# Autodesk Inventor assembly: general
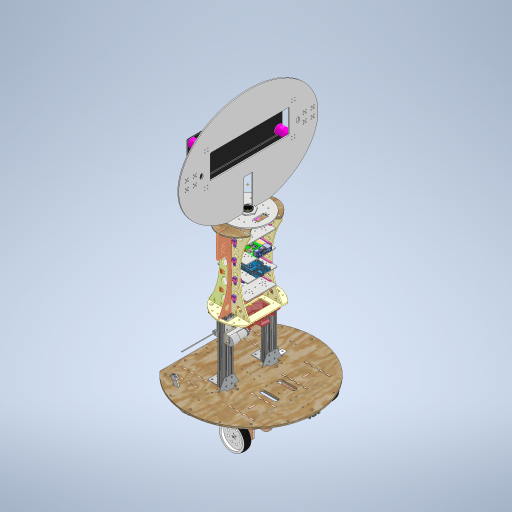
[picture p0: Inventor's stored thumbnail of the model, 512x512]
Saved by Autodesk Inventor 2023.1 (Build 271208000, 208)
## iProperties
Created: 2024-12-19
Part Number: general
Document SubType Name: Assembly
Designer: DELL
Author: DELL
## Documents named in this file (5)
- C:\Users\DELL\reposGitHub\Cheburashka\Cheburashka_construction\general.iam
- C:\Users\DELL\reposGitHub\Cheburashka\Cheburashka_construction\platform\platform.iam
- C:\Users\DELL\reposGitHub\Cheburashka\Cheburashka_construction\korpus\korp.iam
- C:\Users\DELL\reposGitHub\Cheburashka\Cheburashka_construction\platform\8bc17c1464c21f56fb2a3979b7c6b729.ipt
- C:\Users\DELL\reposGitHub\Cheburashka\Cheburashka_construction\face\лицо\Сборка1.iam
## Components (5 placed, 4 different names)
1. platform:1 [sub-assembly] — Заподлицо:1, Совмещение:7, Совмещение:8, Совмещение:13, Совмещение:14
2. korp:1 [sub-assembly] — Заподлицо:1, Совмещение:6, Совмещение:12, Совмещение:15, Совмещение:16, Совмещение:17
3. 8bc17c1464c21f56fb2a3979b7c6b729:2 — Совмещение:6, Совмещение:7, Совмещение:8
4. 8bc17c1464c21f56fb2a3979b7c6b729:4 — Совмещение:12, Совмещение:13, Совмещение:14
5. face [sub-assembly] — Совмещение:15, Совмещение:16, Совмещение:17
## Relationships (10: Mate 9, Flush 1)
- Заподлицо:1 [Flush]: platform:1 ↔ korp:1
- Совмещение:6 [Mate]: korp:1 ↔ 8bc17c1464c21f56fb2a3979b7c6b729:2
- Совмещение:7 [Mate]: platform:1 ↔ 8bc17c1464c21f56fb2a3979b7c6b729:2
- Совмещение:8 [Mate]: platform:1 ↔ 8bc17c1464c21f56fb2a3979b7c6b729:2
- Совмещение:12 [Mate]: korp:1 ↔ 8bc17c1464c21f56fb2a3979b7c6b729:4
- Совмещение:13 [Mate]: platform:1 ↔ 8bc17c1464c21f56fb2a3979b7c6b729:4
- Совмещение:14 [Mate]: platform:1 ↔ 8bc17c1464c21f56fb2a3979b7c6b729:4
- Совмещение:15 [Mate]: korp:1 ↔ face
- Совмещение:16 [Mate]: korp:1 ↔ face
- Совмещение:17 [Mate]: korp:1 ↔ face
